# Autodesk Inventor assembly: !first_stage
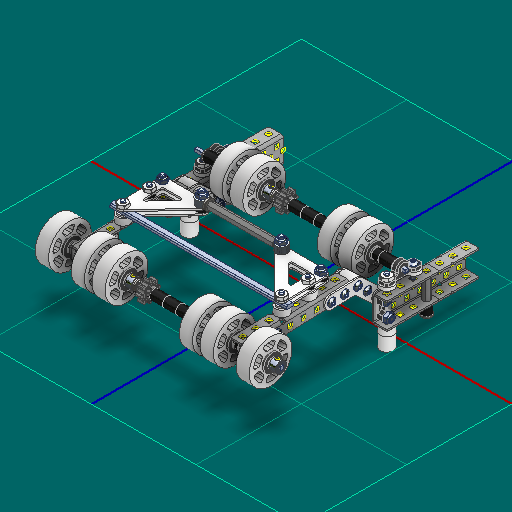
[picture p0: Inventor's stored thumbnail of the model, 512x512]
Saved by Autodesk Inventor 2025 (Build 290162000, 162)
## iProperties
Created: 2024-08-18
Part Number: !first_stage
Document SubType Name: Assembly
Designer: averey
Author: averey
## Documents named in this file (5)
- C:\Users\avere\vex_robotics_high_stakes\hardware\cad\ATLAS\intake\first_stage\!first_stage.iam
- C:\Users\avere\vex_robotics_high_stakes\hardware\cad\ATLAS\intake\first_stage\structure.iam
- C:\Users\avere\vex_robotics_high_stakes\hardware\cad\ATLAS\intake\first_stage\arm\!arm.iam
- C:\Users\avere\vex_robotics_high_stakes\hardware\cad\ATLAS\intake\first_stage\arm\bottom_roller.iam
- C:\Users\avere\vex_robotics_high_stakes\hardware\cad\ATLAS\intake\first_stage\top_roller.iam
## Components (4 placed, 4 different names)
1. structure:1 [sub-assembly] — Mate:2, Insert:2, Insert:3
2. !arm:1 [sub-assembly] — Mate:2, Insert:1, Insert:3
3. bottom_roller:1 [sub-assembly] — Insert:1
4. top_roller:1 [sub-assembly] — Insert:2
## Relationships (4: Insert 3, Mate 1)
- Mate:2: structure:1 ↔ !arm:1
- Insert:1 (6.35 mm): !arm:1 ↔ bottom_roller:1
- Insert:2: structure:1 ↔ top_roller:1
- Insert:3 (0.3969 mm): structure:1 ↔ !arm:1
